# Autodesk Inventor assembly: Prueba
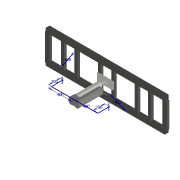
[picture p0: Inventor's stored thumbnail of the model, 180x180]
Saved by Autodesk Inventor 2021 (Build 250183000, 183)
## iProperties
Created: 2021-05-04
Part Number: Prueba
Document SubType Name: Assembly
Designer: Santiago Suárez
Author: Santiago Suárez
## Documents named in this file (8)
- C:\Users\Santiago Suárez\Documents\GitHub\Dis.-Mecatronico-E6\inventor proyecto\Prueba.iam
- C:\Users\Santiago Suárez\Documents\GitHub\Dis.-Mecatronico-E6\inventor proyecto\cilindro\cilindro.iam
- C:\Users\Santiago Suárez\Documents\GitHub\Dis.-Mecatronico-E6\inventor proyecto\Motor1.ipt
- C:\Users\Santiago Suárez\Documents\GitHub\Dis.-Mecatronico-E6\inventor proyecto\manivela.ipt
- C:\Users\Santiago Suárez\Documents\GitHub\Dis.-Mecatronico-E6\inventor proyecto\Biela.ipt
- C:\Users\Santiago Suárez\Documents\GitHub\Dis.-Mecatronico-E6\inventor proyecto\Eje.ipt
- C:\Users\Santiago Suárez\Documents\GitHub\Dis.-Mecatronico-E6\inventor proyecto\marco\Frame\Frame 1618182230761.iam
- C:\Users\Santiago Suárez\Documents\GitHub\Dis.-Mecatronico-E6\inventor proyecto\placa centro.ipt
## Components (10 placed, 7 different names)
1. cilindro:1 [sub-assembly] — Mate:1, Mate:4, Mate:5, Mate:6
2. Motor1:1 — Mate:1, Rotational:1, Rotational:2
3. manivela:1 — Rigid:2, Ball:1
4. manivela:2 — Rigid:1, Ball:2
5. Biela:1 — Ball:2
6. Biela:2 — Ball:1
7. Eje:1 — Rotational:1, Rigid:1
8. Eje:2 — Rotational:2, Rigid:2
9. Frame 1618182230761:1 [sub-assembly] — Mate:2, Mate:3
10. placa centro:1 — Mate:2, Mate:3, Mate:4, Mate:5, Mate:6
## Relationships (12: Mate 6, RevoluteJoint 2, WeldJoint 2, BallJoint 2)
- Mate:1: cilindro:1 ↔ Motor1:1
- Rotational:1 [RevoluteJoint]: Motor1:1 ↔ Eje:1
- Rotational:2 [RevoluteJoint]: Motor1:1 ↔ Eje:2
- Rigid:1 [WeldJoint]: manivela:2 ↔ Eje:1
- Rigid:2 [WeldJoint]: manivela:1 ↔ Eje:2
- Ball:1: manivela:1 ↔ Biela:2
- Ball:2: manivela:2 ↔ Biela:1
- Mate:2: Frame 1618182230761:1 ↔ placa centro:1
- Mate:3 (156 mm): Frame 1618182230761:1 ↔ placa centro:1
- Mate:4: cilindro:1 ↔ placa centro:1
- Mate:5 (42 mm): cilindro:1 ↔ placa centro:1
- Mate:6 (105 mm): cilindro:1 ↔ placa centro:1
